# Autodesk Inventor assembly: Hopper Bottom assy
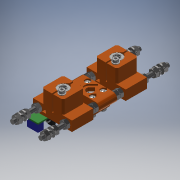
[picture p0: Inventor's stored thumbnail of the model, 180x180]
Saved by Autodesk Inventor 2018 (Build 220112000, 112)
## iProperties
Created: 2017-11-14
Part Number: Hopper Bottom assy
Document SubType Name: Assembly
Designer: Gabriel Smolnycki
Author: Gabriel Smolnycki
## Documents named in this file (7)
- E:\planb\mechanics\V1INV\Subassemblies\Hopper Bottom assy.iam
- E:\planb\mechanics\V1INV\Subassemblies\Hopper Nut Trap assy.iam
- E:\planb\mechanics\V1INV\Hardware\M6 SS Nut.ipt
- E:\planb\mechanics\V1INV\Subassemblies\Hopper Linear Guide assy.iam
- E:\planb\mechanics\V1INV\Subassemblies\Hopper Linear Guide with endstop assy.iam
- E:\planb\mechanics\V1INV\Hopper\Hopper M6 rod.ipt
- E:\planb\mechanics\V1INV\Hardware\M6 SS Washer.ipt
## Components (33 placed, 6 different names)
1. Hopper Nut Trap assy:1 [sub-assembly] — Insert:1, Insert:3, Insert:5, Insert:7, Flush:1, Flush:2, Flush:3, Flush:4, Mate:1, Mate:2
2. M6 SS Nut:1 — Insert:1, Insert:2
3. M6 SS Nut:2 — Insert:2, Insert:12
4. M6 SS Nut:3 — Insert:6, Insert:9
5. M6 SS Nut:4 — Insert:5, Insert:6
6. M6 SS Nut:5 — Insert:3, Insert:4
7. M6 SS Nut:6 — Insert:4, Insert:11
8. M6 SS Nut:7 — Insert:8, Insert:10
9. M6 SS Nut:8 — Insert:7, Insert:8
10. Hopper Linear Guide assy:1 [sub-assembly] — Insert:9, Insert:10, Insert:15, Insert:16
11. Hopper Linear Guide with endstop assy:1 [sub-assembly] — Insert:11, Insert:12, Insert:13, Insert:14
12. M6 SS Nut:9 — Insert:13, Insert:22
13. M6 SS Nut:10 — Insert:14, Insert:21
14. M6 SS Nut:11 — Insert:15, Insert:18, Insert:19
15. M6 SS Nut:12 — Insert:16, Insert:17, Insert:20
16. Hopper M6 rod:1 — Flush:2, Insert:18
17. Hopper M6 rod:2 — Flush:1, Insert:17
18. M6 SS Washer:1 — Flush:4, Insert:20, Insert:26, Insert:30
19. M6 SS Washer:2 — Flush:3, Insert:19, Insert:25, Insert:29
20. M6 SS Washer:3 — Mate:2, Insert:21, Insert:23, Insert:27
21. M6 SS Washer:4 — Mate:1, Insert:22, Insert:24, Insert:28
22. M6 SS Nut:13 — Insert:23
23. M6 SS Nut:14 — Insert:24
24. M6 SS Nut:15 — Insert:26
25. M6 SS Nut:16 — Insert:25
26. M6 SS Washer:5 — Insert:28, Insert:33
27. M6 SS Washer:6 — Insert:27, Insert:34
28. M6 SS Washer:7 — Insert:29, Insert:32
29. M6 SS Washer:8 — Insert:30, Insert:31
30. M6 SS Nut:17 — Insert:31
31. M6 SS Nut:18 — Insert:32
32. M6 SS Nut:19 — Insert:33
33. M6 SS Nut:20 — Insert:34
## Relationships (40: Insert 34, Flush 4, Mate 2)
- Insert:1: Hopper Nut Trap assy:1 ↔ M6 SS Nut:1
- Insert:2 (0.5 mm): M6 SS Nut:1 ↔ M6 SS Nut:2
- Insert:3: Hopper Nut Trap assy:1 ↔ M6 SS Nut:5
- Insert:4 (0.5 mm): M6 SS Nut:5 ↔ M6 SS Nut:6
- Insert:5: Hopper Nut Trap assy:1 ↔ M6 SS Nut:4
- Insert:6 (0.5 mm): M6 SS Nut:3 ↔ M6 SS Nut:4
- Insert:7: Hopper Nut Trap assy:1 ↔ M6 SS Nut:8
- Insert:8 (0.5 mm): M6 SS Nut:7 ↔ M6 SS Nut:8
- Insert:9: M6 SS Nut:3 ↔ Hopper Linear Guide assy:1
- Insert:10: M6 SS Nut:7 ↔ Hopper Linear Guide assy:1
- Insert:11: M6 SS Nut:6 ↔ Hopper Linear Guide with endstop assy:1
- Insert:12: M6 SS Nut:2 ↔ Hopper Linear Guide with endstop assy:1
- Insert:13: Hopper Linear Guide with endstop assy:1 ↔ M6 SS Nut:9
- Insert:14: Hopper Linear Guide with endstop assy:1 ↔ M6 SS Nut:10
- Insert:15: Hopper Linear Guide assy:1 ↔ M6 SS Nut:11
- Insert:16: Hopper Linear Guide assy:1 ↔ M6 SS Nut:12
- Flush:1 (90 mm): Hopper Nut Trap assy:1 ↔ Hopper M6 rod:2
- Flush:2 (90 mm): Hopper Nut Trap assy:1 ↔ Hopper M6 rod:1
- Insert:17: M6 SS Nut:12 ↔ Hopper M6 rod:2
- Insert:18: M6 SS Nut:11 ↔ Hopper M6 rod:1
- Flush:3 (75 mm): Hopper Nut Trap assy:1 ↔ M6 SS Washer:2
- Flush:4 (75 mm): Hopper Nut Trap assy:1 ↔ M6 SS Washer:1
- Insert:19: M6 SS Nut:11 ↔ M6 SS Washer:2
- Insert:20: M6 SS Nut:12 ↔ M6 SS Washer:1
- Mate:1 (-75 mm): Hopper Nut Trap assy:1 ↔ M6 SS Washer:4
- Mate:2 (-75 mm): Hopper Nut Trap assy:1 ↔ M6 SS Washer:3
- Insert:21: M6 SS Nut:10 ↔ M6 SS Washer:3
- Insert:22: M6 SS Nut:9 ↔ M6 SS Washer:4
- Insert:23: M6 SS Washer:3 ↔ M6 SS Nut:13
- Insert:24: M6 SS Washer:4 ↔ M6 SS Nut:14
- Insert:25: M6 SS Washer:2 ↔ M6 SS Nut:16
- Insert:26: M6 SS Washer:1 ↔ M6 SS Nut:15
- Insert:27 (4.064 mm): M6 SS Washer:3 ↔ M6 SS Washer:6
- Insert:28 (4.064 mm): M6 SS Washer:4 ↔ M6 SS Washer:5
- Insert:29 (4.064 mm): M6 SS Washer:2 ↔ M6 SS Washer:7
- Insert:30 (4.064 mm): M6 SS Washer:1 ↔ M6 SS Washer:8
- Insert:31: M6 SS Washer:8 ↔ M6 SS Nut:17
- Insert:32: M6 SS Washer:7 ↔ M6 SS Nut:18
- Insert:33: M6 SS Washer:5 ↔ M6 SS Nut:19
- Insert:34: M6 SS Washer:6 ↔ M6 SS Nut:20
